# Autodesk Inventor assembly: Structure
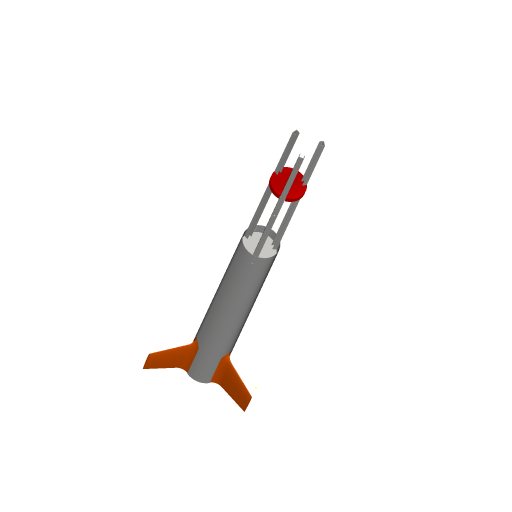
[picture p0: Inventor's stored thumbnail of the model, 512x512]
Saved by Autodesk Inventor 2024 (Build 280153000, 153)
## iProperties
Created: 2023-12-30
Part Number: Structure
Document SubType Name: Assembly
Designer: Jamie
Mass: 490.976 g
Surface Area: 3690.03 cm^2
Volume: 269.832 cm^3
Density: 1.81956 g/cm^3
Author: Jamie
## Documents named in this file (6)
- C:\Users\Jamie\Documents\Uni\DARE\Scrambler-2-CAD\Autodesk\Structure.iam
- C:\Users\Jamie\Documents\Uni\DARE\Scrambler-2-CAD\Autodesk\Engine bulkhead.ipt
- C:\Users\Jamie\Documents\Uni\DARE\Scrambler-2-CAD\Autodesk\Stringer.ipt
- C:\Users\Jamie\Documents\Uni\DARE\Scrambler-2-CAD\Autodesk\Parachute bulkhead.ipt
- C:\Users\Jamie\Documents\Uni\DARE\Scrambler-2-CAD\Autodesk\Engine skin glued.iam
- Engine skin.iam
## Components (6 placed, 4 different names)
1. Engine bulkhead:1 — Mate:26, Mate:27
2. Stringer:1 — Mate:12, Mate:23, Mate:29
3. Stringer:2 — Mate:13, Mate:15, Mate:30
4. Stringer:3 — Mate:11, Mate:25, Mate:28
5. Parachute bulkhead:1 — Mate:11, Mate:12, Mate:13, Mate:15, Mate:23, Mate:25
6. Engine skin:1 [sub-assembly] — Mate:26, Mate:27, Mate:28, Mate:29, Mate:30
## Relationships (11: Mate 11)
- Mate:11 (0.5 mm): Stringer:3 ↔ Parachute bulkhead:1
- Mate:12 (0.5 mm): Stringer:1 ↔ Parachute bulkhead:1
- Mate:13 (0.5 mm): Stringer:2 ↔ Parachute bulkhead:1
- Mate:15: Stringer:2 ↔ Parachute bulkhead:1
- Mate:23: Stringer:1 ↔ Parachute bulkhead:1
- Mate:25: Stringer:3 ↔ Parachute bulkhead:1
- Mate:26: Engine bulkhead:1 ↔ Engine skin:1
- Mate:27: Engine bulkhead:1 ↔ Engine skin:1
- Mate:28: Stringer:3 ↔ Engine skin:1
- Mate:29: Stringer:1 ↔ Engine skin:1
- Mate:30: Stringer:2 ↔ Engine skin:1
